# Autodesk Inventor assembly: Full Cartridge Interface
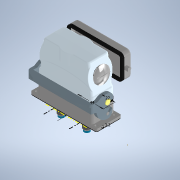
[picture p0: Inventor's stored thumbnail of the model, 180x180]
Saved by Autodesk Inventor 2021 (Build 250183000, 183)
## iProperties
Created: 2020-04-03
Part Number: Full Cartridge Interface
Document SubType Name: Assembly
Designer: jgray
Author: jgray
## Documents named in this file (8)
- M:\Printed Electronics\Gas Sensors\Prototypes\Prototype II -Cartridge Reader V3\Full Cartridge Interface.iam
- M:\Printed Electronics\Gas Sensors\Prototypes\Prototype II -Cartridge Reader V3\KCE04-00(5-3)_BU_BODY.ipt
- M:\Printed Electronics\Gas Sensors\Prototypes\Prototype II -Cartridge Reader V3\Cartridge Clamp1771613.iam
- M:\Printed Electronics\Gas Sensors\Prototypes\Prototype II -Cartridge Reader V3\Cartridge Full.iam
- M:\Printed Electronics\Gas Sensors\Prototypes\Prototype II -Cartridge Reader V3\InterfaceBlock-OutPCB-Connectors.iam
- M:\Printed Electronics\Gas Sensors\Prototypes\Prototype II -Cartridge Reader V3\DIN 6798 - J 3.2.ipt
- M:\Printed Electronics\Gas Sensors\Prototypes\Prototype II -Cartridge Reader V3\DIN 7985 (H) - M3x22-H.ipt
- M:\Printed Electronics\Gas Sensors\Prototypes\Prototype II -Cartridge Reader V3\DIN 934 - M3 x 0.5.ipt
## Components (21 placed, 7 different names)
1. KCE04-00(5-3)_BU_BODY:1 — Flush:1, Mate:10, Mate:15
2. KCE04-00(5-3)_BU_BODY:2 — Flush:1, Mate:11, Flush:2, Mate:16
3. Cartridge Clamp1771613:1 [sub-assembly] — Mate:8, Mate:9, Mate:12, Mate:13, Mate:14, Mate:17, Mate:30, Mate:31, Mate:32, Mate:33, Mate:34, Mate:35, Mate:36, Mate:37
4. Cartridge Full:1 [sub-assembly] — Mate:15, Mate:16, Mate:17
5. InterfaceBlock-OutPCB-Connectors:1 [sub-assembly] — Mate:10, Mate:11, Flush:2, Mate:12, Mate:13, Mate:14, Mate:26, Mate:27, Mate:28, Mate:29
6. DIN 6798 J J 3.2:1 — Mate:18, Mate:25, Mate:29
7. DIN 6798 J J 3.2:2 — Mate:19, Mate:23, Mate:27
8. DIN 6798 J J 3.2:3 — Mate:20, Mate:24, Mate:26
9. DIN 6798 J J 3.2:4 — Mate:21, Mate:22, Mate:28
10. DIN 6798 J J 3.2:5 — Mate:37, Mate:41, Mate:44
11. DIN 6798 J J 3.2:6 — Mate:35, Mate:39, Mate:45
12. DIN 6798 J J 3.2:7 — Mate:36, Mate:40, Mate:42
13. DIN 6798 J J 3.2:8 — Mate:34, Mate:38, Mate:43
14. DIN 7985 (H) M3x22-H:1 — Mate:21, Mate:22, Mate:33, Mate:38, Mate:47
15. DIN 7985 (H) M3x22-H:2 — Mate:19, Mate:23, Mate:30, Mate:41, Mate:48
16. DIN 7985 (H) M3x22-H:3 — Mate:20, Mate:24, Mate:31, Mate:40, Mate:49
17. DIN 7985 (H) M3x22-H:4 — Mate:18, Mate:25, Mate:32, Mate:39, Mate:46
18. DIN 934 - replaced by DIN EN 24032/28673/28674 M3:1 — Mate:43, Mate:47
19. DIN 934 - replaced by DIN EN 24032/28673/28674 M3:2 — Mate:45, Mate:46
20. DIN 934 - replaced by DIN EN 24032/28673/28674 M3:3 — Mate:42, Mate:49
21. DIN 934 - replaced by DIN EN 24032/28673/28674 M3:4 — Mate:44, Mate:48
## Relationships (44: Mate 42, Flush 2)
- Flush:1: KCE04-00(5-3)_BU_BODY:1 ↔ KCE04-00(5-3)_BU_BODY:2
- Mate:8: Cartridge Clamp1771613:1
- Mate:9: Cartridge Clamp1771613:1
- Mate:10: KCE04-00(5-3)_BU_BODY:1 ↔ InterfaceBlock-OutPCB-Connectors:1
- Mate:11: KCE04-00(5-3)_BU_BODY:2 ↔ InterfaceBlock-OutPCB-Connectors:1
- Flush:2: KCE04-00(5-3)_BU_BODY:2 ↔ InterfaceBlock-OutPCB-Connectors:1
- Mate:12: Cartridge Clamp1771613:1 ↔ InterfaceBlock-OutPCB-Connectors:1
- Mate:13: Cartridge Clamp1771613:1 ↔ InterfaceBlock-OutPCB-Connectors:1
- Mate:14: Cartridge Clamp1771613:1 ↔ InterfaceBlock-OutPCB-Connectors:1
- Mate:15: KCE04-00(5-3)_BU_BODY:1 ↔ Cartridge Full:1
- Mate:16: KCE04-00(5-3)_BU_BODY:2 ↔ Cartridge Full:1
- Mate:17 (-0.62 mm): Cartridge Clamp1771613:1 ↔ Cartridge Full:1
- Mate:18: DIN 6798 J J 3.2:1 ↔ DIN 7985 (H) M3x22-H:4
- Mate:19: DIN 6798 J J 3.2:2 ↔ DIN 7985 (H) M3x22-H:2
- Mate:20: DIN 6798 J J 3.2:3 ↔ DIN 7985 (H) M3x22-H:3
- Mate:21: DIN 6798 J J 3.2:4 ↔ DIN 7985 (H) M3x22-H:1
- Mate:22: DIN 6798 J J 3.2:4 ↔ DIN 7985 (H) M3x22-H:1
- Mate:23: DIN 6798 J J 3.2:2 ↔ DIN 7985 (H) M3x22-H:2
- Mate:24: DIN 6798 J J 3.2:3 ↔ DIN 7985 (H) M3x22-H:3
- Mate:25: DIN 6798 J J 3.2:1 ↔ DIN 7985 (H) M3x22-H:4
- Mate:26: InterfaceBlock-OutPCB-Connectors:1 ↔ DIN 6798 J J 3.2:3
- Mate:27: InterfaceBlock-OutPCB-Connectors:1 ↔ DIN 6798 J J 3.2:2
- Mate:28: InterfaceBlock-OutPCB-Connectors:1 ↔ DIN 6798 J J 3.2:4
- Mate:29: InterfaceBlock-OutPCB-Connectors:1 ↔ DIN 6798 J J 3.2:1
- Mate:30: Cartridge Clamp1771613:1 ↔ DIN 7985 (H) M3x22-H:2
- Mate:31: Cartridge Clamp1771613:1 ↔ DIN 7985 (H) M3x22-H:3
- Mate:32: Cartridge Clamp1771613:1 ↔ DIN 7985 (H) M3x22-H:4
- Mate:33: Cartridge Clamp1771613:1 ↔ DIN 7985 (H) M3x22-H:1
- Mate:34: Cartridge Clamp1771613:1 ↔ DIN 6798 J J 3.2:8
- Mate:35: Cartridge Clamp1771613:1 ↔ DIN 6798 J J 3.2:6
- Mate:36: Cartridge Clamp1771613:1 ↔ DIN 6798 J J 3.2:7
- Mate:37: Cartridge Clamp1771613:1 ↔ DIN 6798 J J 3.2:5
- Mate:38: DIN 6798 J J 3.2:8 ↔ DIN 7985 (H) M3x22-H:1
- Mate:39: DIN 6798 J J 3.2:6 ↔ DIN 7985 (H) M3x22-H:4
- Mate:40: DIN 6798 J J 3.2:7 ↔ DIN 7985 (H) M3x22-H:3
- Mate:41: DIN 6798 J J 3.2:5 ↔ DIN 7985 (H) M3x22-H:2
- Mate:42: DIN 6798 J J 3.2:7 ↔ DIN 934 - replaced by DIN EN 24032/28673/28674 M3:3
- Mate:43: DIN 6798 J J 3.2:8 ↔ DIN 934 - replaced by DIN EN 24032/28673/28674 M3:1
- Mate:44: DIN 6798 J J 3.2:5 ↔ DIN 934 - replaced by DIN EN 24032/28673/28674 M3:4
- Mate:45: DIN 6798 J J 3.2:6 ↔ DIN 934 - replaced by DIN EN 24032/28673/28674 M3:2
- Mate:46: DIN 7985 (H) M3x22-H:4 ↔ DIN 934 - replaced by DIN EN 24032/28673/28674 M3:2
- Mate:47: DIN 7985 (H) M3x22-H:1 ↔ DIN 934 - replaced by DIN EN 24032/28673/28674 M3:1
- Mate:48: DIN 7985 (H) M3x22-H:2 ↔ DIN 934 - replaced by DIN EN 24032/28673/28674 M3:4
- Mate:49: DIN 7985 (H) M3x22-H:3 ↔ DIN 934 - replaced by DIN EN 24032/28673/28674 M3:3
